# Autodesk Inventor assembly: Brazo
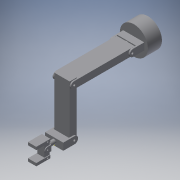
[picture p0: Inventor's stored thumbnail of the model, 180x180]
Saved by Autodesk Inventor 2019 (Build 230136000, 136)
## iProperties
Created: 2019-10-18
Part Number: Brazo
Material: Genérico
Document SubType Name: Assembly
Designer: Josue
Author: Josue
## Documents named in this file (7)
- C:\Users\Josue\OneDrive\Escritorio\Inverto\Brazo.iam
- C:\Users\Josue\OneDrive\Escritorio\Inverto\base redonda.ipt
- C:\Users\Josue\OneDrive\Escritorio\Inverto\primer rotor.ipt
- C:\Users\Josue\OneDrive\Escritorio\Inverto\brazo 1.ipt
- C:\Users\Josue\OneDrive\Escritorio\Inverto\brazo2.ipt
- C:\Users\Josue\OneDrive\Escritorio\Inverto\Muñeca.ipt
- C:\Users\Josue\OneDrive\Escritorio\Inverto\pinza.ipt
## Components (6 placed, 6 different names)
1. base redonda:1 — Coincidencia:1
2. primer rotor:1 — Coincidencia:1, Coincidencia:2
3. brazo 1:1 — Coincidencia:2, Coincidencia:3
4. brazo2:1 — Coincidencia:3
5. Muñeca:1 — De rotación:1
6. pinza:1 — De rotación:1
## Relationships (4: Mate 3, RevoluteJoint 1)
- Coincidencia:1 [Mate]: base redonda:1 ↔ primer rotor:1
- Coincidencia:2 [Mate] (3.454 mm): primer rotor:1 ↔ brazo 1:1
- Coincidencia:3 [Mate]: brazo 1:1 ↔ brazo2:1
- De rotación:1 [RevoluteJoint]: Muñeca:1 ↔ pinza:1
